# Autodesk Inventor assembly: Klick-00_Xol_D2F_PCB _1__MIR
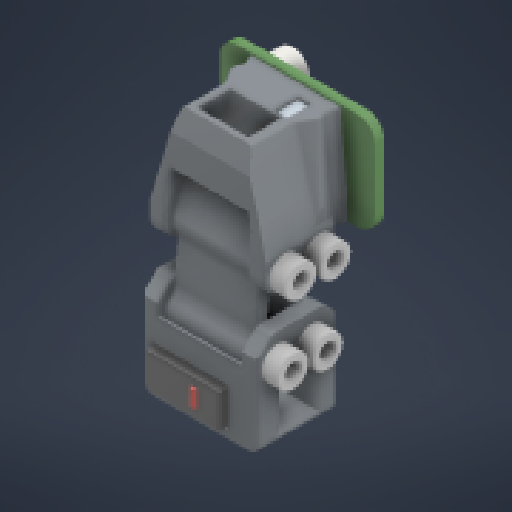
[picture p0: Inventor's stored thumbnail of the model, 512x512]
Saved by Autodesk Inventor 2024.3 (Build 283343000, 343)
## iProperties
Created: 2024-12-01
Part Number: Klick-00_Xol_D2F_PCB _1__MIR
Document SubType Name: Assembly
Designer: MFil
Author: MFil
## Documents named in this file (11)
- C:\ROBOTYKA\myVORON tridex\Hotend carriges\parts\Klicky-00 - RC2 Assemblies\Klicky-00 - RC2 Assemblies\Klick-00_Xol_D2F_PCB _1__MIR.iam
- C:\ROBOTYKA\myVORON tridex\Hotend carriges\parts\Klicky-00 - RC2 Assemblies\Klicky-00 - RC2 Assemblies\Magnet [6x3]_MIR.ipt
- C:\ROBOTYKA\myVORON tridex\Hotend carriges\parts\Klicky-00 - RC2 Assemblies\Klicky-00 - RC2 Assemblies\Klicky-00_PCB_Klicky_Rear_MIR.ipt
- C:\ROBOTYKA\myVORON tridex\Hotend carriges\parts\Klicky-00 - RC2 Assemblies\Klicky-00 - RC2 Assemblies\Klicky-00_Xol_PCB_Swingarm_Upper_MIR.ipt
- C:\ROBOTYKA\myVORON tridex\Hotend carriges\parts\Klicky-00 - RC2 Assemblies\Klicky-00 - RC2 Assemblies\D2F_ACTUATOR_MIR.ipt
- C:\ROBOTYKA\myVORON tridex\Hotend carriges\parts\Klicky-00 - RC2 Assemblies\Klicky-00 - RC2 Assemblies\M2x10 FHCS self tapping screw_MIR.ipt
- C:\ROBOTYKA\myVORON tridex\Hotend carriges\parts\Klicky-00 - RC2 Assemblies\Klicky-00 - RC2 Assemblies\Klicky-00_Xol_PCB_Swingarm_Lower_MIR.ipt
- C:\ROBOTYKA\myVORON tridex\Hotend carriges\parts\Klicky-00 - RC2 Assemblies\Klicky-00 - RC2 Assemblies\M3x20 SHCS_MIR.ipt
- C:\ROBOTYKA\myVORON tridex\Hotend carriges\parts\Klicky-00 - RC2 Assemblies\Klicky-00 - RC2 Assemblies\D2F_BASE_MIR.ipt
- C:\ROBOTYKA\myVORON tridex\Hotend carriges\parts\Klicky-00 - RC2 Assemblies\Klicky-00 - RC2 Assemblies\Klicky-00_Xol_D2F_Front_MIR.ipt
- C:\ROBOTYKA\myVORON tridex\Hotend carriges\parts\Klicky-00 - RC2 Assemblies\Klicky-00 - RC2 Assemblies\PCB-Klicky_Probe-side _1_ (2)_MIR.iam
## Components (17 placed, 10 different names)
1. Magnet [6x3]_MIR:1 — Mate:18, Mate:17
2. Klicky-00_PCB_Klicky_Rear_MIR:1 — Mate:15, Mate:13, Mate:8, Mate:7, Mate:12, Mate:16, Mate:14, Mate:11, Flush:6, Mate:4, Mate:3, Mate:2, Mate:1, Mate:6, Mate:5
3. Klicky-00_Xol_PCB_Swingarm_Upper_MIR:1 — Mate:15, Mate:13, Flush:1, Mate:20, Mate:19
4. D2F_ACTUATOR_MIR:1 — Mate:31, Mate:30, Mate:29
5. Magnet [6x3]_MIR:2 — Mate:10, Mate:9
6. Magnet [6x3]_MIR:3 — Mate:8, Mate:7
7. M2x10 FHCS self tapping screw_MIR:1 — Flush:4, Flush:5, Mate:27
8. Klicky-00_Xol_PCB_Swingarm_Lower_MIR:1 — Flush:1, Mate:12, Mate:10, Mate:9, Mate:21
9. M3x20 SHCS_MIR:1 — Mate:16, Mate:14, Flush:2
10. M3x20 SHCS_MIR:2 — Flush:2, Mate:11
11. D2F_BASE_MIR:1 — Mate:31, Mate:30, Mate:29, Mate:32, Mate:26, Mate:25
12. M3x20 SHCS_MIR:3 — Mate:23, Flush:3
13. M2x10 FHCS self tapping screw_MIR:2 — Flush:4, Mate:28
14. Klicky-00_Xol_D2F_Front_MIR:1 — Flush:6, Mate:32, Flush:5, Mate:28, Mate:27, Mate:26, Mate:25, Mate:23, Mate:21, Mate:20, Mate:19, Mate:18, Mate:17, Mate:24, Mate:22, Flush:7
15. M3x20 SHCS_MIR:4 — Mate:24, Flush:3, Mate:22
16. PCB-Klicky_Probe-side _1_ (2)_MIR:1 [sub-assembly] — Mate:4, Mate:3, Mate:2, Mate:1, Flush:7
17. Magnet [6x3]_MIR:4 — Mate:6, Mate:5
## Relationships (39: Mate 32, Flush 7)
- Mate:15 (0.1 mm): Klicky-00_PCB_Klicky_Rear_MIR:1 ↔ Klicky-00_Xol_PCB_Swingarm_Upper_MIR:1
- Mate:13: Klicky-00_PCB_Klicky_Rear_MIR:1 ↔ Klicky-00_Xol_PCB_Swingarm_Upper_MIR:1
- Mate:8: Klicky-00_PCB_Klicky_Rear_MIR:1 ↔ Magnet [6x3]_MIR:3
- Mate:7: Klicky-00_PCB_Klicky_Rear_MIR:1 ↔ Magnet [6x3]_MIR:3
- Flush:1: Klicky-00_Xol_PCB_Swingarm_Upper_MIR:1 ↔ Klicky-00_Xol_PCB_Swingarm_Lower_MIR:1
- Mate:12: Klicky-00_PCB_Klicky_Rear_MIR:1 ↔ Klicky-00_Xol_PCB_Swingarm_Lower_MIR:1
- Mate:10: Magnet [6x3]_MIR:2 ↔ Klicky-00_Xol_PCB_Swingarm_Lower_MIR:1
- Mate:9: Magnet [6x3]_MIR:2 ↔ Klicky-00_Xol_PCB_Swingarm_Lower_MIR:1
- Mate:16: Klicky-00_PCB_Klicky_Rear_MIR:1 ↔ M3x20 SHCS_MIR:1
- Mate:14: Klicky-00_PCB_Klicky_Rear_MIR:1 ↔ M3x20 SHCS_MIR:1
- Flush:2: M3x20 SHCS_MIR:1 ↔ M3x20 SHCS_MIR:2
- Mate:11: Klicky-00_PCB_Klicky_Rear_MIR:1 ↔ M3x20 SHCS_MIR:2
- Mate:31: D2F_ACTUATOR_MIR:1 ↔ D2F_BASE_MIR:1
- Mate:30: D2F_ACTUATOR_MIR:1 ↔ D2F_BASE_MIR:1
- Mate:29: D2F_ACTUATOR_MIR:1 ↔ D2F_BASE_MIR:1
- Flush:4: M2x10 FHCS self tapping screw_MIR:1 ↔ M2x10 FHCS self tapping screw_MIR:2
- Flush:6: Klicky-00_PCB_Klicky_Rear_MIR:1 ↔ Klicky-00_Xol_D2F_Front_MIR:1
- Mate:32 (0.15 mm): D2F_BASE_MIR:1 ↔ Klicky-00_Xol_D2F_Front_MIR:1
- Flush:5: M2x10 FHCS self tapping screw_MIR:1 ↔ Klicky-00_Xol_D2F_Front_MIR:1
- Mate:28: M2x10 FHCS self tapping screw_MIR:2 ↔ Klicky-00_Xol_D2F_Front_MIR:1
- Mate:27: M2x10 FHCS self tapping screw_MIR:1 ↔ Klicky-00_Xol_D2F_Front_MIR:1
- Mate:26: D2F_BASE_MIR:1 ↔ Klicky-00_Xol_D2F_Front_MIR:1
- Mate:25: D2F_BASE_MIR:1 ↔ Klicky-00_Xol_D2F_Front_MIR:1
- Mate:23: M3x20 SHCS_MIR:3 ↔ Klicky-00_Xol_D2F_Front_MIR:1
- Mate:21: Klicky-00_Xol_PCB_Swingarm_Lower_MIR:1 ↔ Klicky-00_Xol_D2F_Front_MIR:1
- Mate:20: Klicky-00_Xol_PCB_Swingarm_Upper_MIR:1 ↔ Klicky-00_Xol_D2F_Front_MIR:1
- Mate:19 (0.1 mm): Klicky-00_Xol_PCB_Swingarm_Upper_MIR:1 ↔ Klicky-00_Xol_D2F_Front_MIR:1
- Mate:18: Magnet [6x3]_MIR:1 ↔ Klicky-00_Xol_D2F_Front_MIR:1
- Mate:17: Magnet [6x3]_MIR:1 ↔ Klicky-00_Xol_D2F_Front_MIR:1
- Mate:24: Klicky-00_Xol_D2F_Front_MIR:1 ↔ M3x20 SHCS_MIR:4
- Flush:3: M3x20 SHCS_MIR:3 ↔ M3x20 SHCS_MIR:4
- Mate:22: Klicky-00_Xol_D2F_Front_MIR:1 ↔ M3x20 SHCS_MIR:4
- Mate:4: Klicky-00_PCB_Klicky_Rear_MIR:1 ↔ PCB-Klicky_Probe-side _1_ (2)_MIR:1
- Mate:3: Klicky-00_PCB_Klicky_Rear_MIR:1 ↔ PCB-Klicky_Probe-side _1_ (2)_MIR:1
- Mate:2: Klicky-00_PCB_Klicky_Rear_MIR:1 ↔ PCB-Klicky_Probe-side _1_ (2)_MIR:1
- Mate:1: Klicky-00_PCB_Klicky_Rear_MIR:1 ↔ PCB-Klicky_Probe-side _1_ (2)_MIR:1
- Mate:6: Klicky-00_PCB_Klicky_Rear_MIR:1 ↔ Magnet [6x3]_MIR:4
- Mate:5: Klicky-00_PCB_Klicky_Rear_MIR:1 ↔ Magnet [6x3]_MIR:4
- Flush:7 (4 mm): Klicky-00_Xol_D2F_Front_MIR:1 ↔ PCB-Klicky_Probe-side _1_ (2)_MIR:1
